# Autodesk Inventor assembly: CapstonCounterweight_assembly
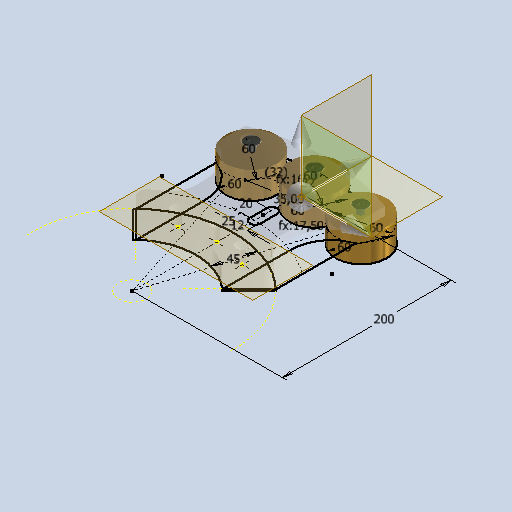
[picture p0: Inventor's stored thumbnail of the model, 512x512]
Saved by Autodesk Inventor 2024 (Build 280153000, 153)
## iProperties
Created: 2022-10-27
Part Number: CapstonCounterweight_assembly
Document SubType Name: Assembly
Designer: alexw
Mass: 2625.33 g
Surface Area: 997.885 cm^2
Volume: 547.099 cm^3
Density: 4.79863 g/cm^3
Author: alexw
## Documents named in this file (6)
- C:\Users\AEWALDER\Documents\Inventor\03_CurrentProjects\MasterThesis\PSM_V1_Rillenkugellager\CapstonCounterweight_assembly.iam
- C:\Users\AEWALDER\Documents\Inventor\03_CurrentProjects\MasterThesis\PSM_V1_Rillenkugellager\CounterweightFixation_Axis0.ipt
- C:\Users\AEWALDER\Documents\Inventor\03_CurrentProjects\MasterThesis\PSM_V1_Rillenkugellager\CapstonAxis0_Weights.ipt
- C:\Users\AEWALDER\Documents\Inventor\03_CurrentProjects\MasterThesis\PSM_V1_Rillenkugellager\ContentCenter\de-DE\ISO 10642(1)\ISO 10642 - M8 x  50.ipt
- C:\Users\AEWALDER\Documents\Inventor\03_CurrentProjects\MasterThesis\PSM_V1_Rillenkugellager\ContentCenter\de-DE\ISO 4032(2)\ISO 4032 - M8 - ISO.ipt
- C:\Users\AEWALDER\Documents\Inventor\03_CurrentProjects\MasterThesis\PSM_V1_Rillenkugellager\ContentCenter\de-DE\ISO 7092\ISO 7092 - ST 8 - 140 HV.ipt
## Components (13 placed, 5 different names)
1. CounterweightFixation_Axis0:1 — Passend:1, Passend:2, Passend:3, Passend:4, Passend:5, Passend:6, Passend:7, Passend:8, Passend:9
2. CapstonAxis0_Weights:1 — Passend:1, Passend:2, Passend:11
3. CapstonAxis0_Weights:2 — Passend:4, Passend:5, Passend:15
4. CapstonAxis0_Weights:3 — Passend:3, Passend:6, Passend:13
5. ISO 10642 M8x50:1 — Passend:7, Passend:14, Passend:20
6. ISO 10642 M8x50:2 — Passend:8, Passend:12, Passend:18
7. ISO 10642 M8x50:3 — Passend:9, Passend:10, Passend:16
8. ISO 7092 ST 8 - 140 HV:1 — Passend:10, Passend:11, Passend:17
9. ISO 7092 ST 8 - 140 HV:2 — Passend:12, Passend:13, Passend:19
10. ISO 7092 ST 8 - 140 HV:3 — Passend:14, Passend:15, Passend:21
11. ISO 4032 M8:1 — Passend:16, Passend:17
12. ISO 4032 M8:2 — Passend:18, Passend:19
13. ISO 4032 M8:3 — Passend:20, Passend:21
## Relationships (21: Mate 21)
- Passend:1 [Mate]: CounterweightFixation_Axis0:1 ↔ CapstonAxis0_Weights:1
- Passend:2 [Mate]: CounterweightFixation_Axis0:1 ↔ CapstonAxis0_Weights:1
- Passend:3 [Mate]: CounterweightFixation_Axis0:1 ↔ CapstonAxis0_Weights:3
- Passend:4 [Mate]: CounterweightFixation_Axis0:1 ↔ CapstonAxis0_Weights:2
- Passend:5 [Mate]: CounterweightFixation_Axis0:1 ↔ CapstonAxis0_Weights:2
- Passend:6 [Mate]: CounterweightFixation_Axis0:1 ↔ CapstonAxis0_Weights:3
- Passend:7 [Mate]: CounterweightFixation_Axis0:1 ↔ ISO 10642 M8x50:1
- Passend:8 [Mate]: CounterweightFixation_Axis0:1 ↔ ISO 10642 M8x50:2
- Passend:9 [Mate]: CounterweightFixation_Axis0:1 ↔ ISO 10642 M8x50:3
- Passend:10 [Mate]: ISO 10642 M8x50:3 ↔ ISO 7092 ST 8 - 140 HV:1
- Passend:11 [Mate]: CapstonAxis0_Weights:1 ↔ ISO 7092 ST 8 - 140 HV:1
- Passend:12 [Mate]: ISO 10642 M8x50:2 ↔ ISO 7092 ST 8 - 140 HV:2
- Passend:13 [Mate]: CapstonAxis0_Weights:3 ↔ ISO 7092 ST 8 - 140 HV:2
- Passend:14 [Mate]: ISO 10642 M8x50:1 ↔ ISO 7092 ST 8 - 140 HV:3
- Passend:15 [Mate]: CapstonAxis0_Weights:2 ↔ ISO 7092 ST 8 - 140 HV:3
- Passend:16 [Mate]: ISO 10642 M8x50:3 ↔ ISO 4032 M8:1
- Passend:17 [Mate]: ISO 7092 ST 8 - 140 HV:1 ↔ ISO 4032 M8:1
- Passend:18 [Mate]: ISO 10642 M8x50:2 ↔ ISO 4032 M8:2
- Passend:19 [Mate]: ISO 7092 ST 8 - 140 HV:2 ↔ ISO 4032 M8:2
- Passend:20 [Mate]: ISO 10642 M8x50:1 ↔ ISO 4032 M8:3
- Passend:21 [Mate]: ISO 7092 ST 8 - 140 HV:3 ↔ ISO 4032 M8:3
